# Autodesk Inventor assembly: 1400_DC Coil_V1
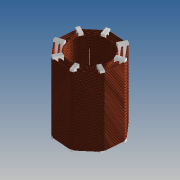
[picture p0: Inventor's stored thumbnail of the model, 180x180]
Saved by Autodesk Inventor 2020 (Build 240168000, 168)
## iProperties
Created: 2019-11-14
Part Number: 1400_DC Coil_V1
Document SubType Name: Assembly
Designer: RFLab
Author: RFLab
## Documents named in this file (6)
- C:\Users\RFLab\Dropbox\MPI Group Folder\MPS\Inventor_Parts\Parts Numbered - OSMPI\1xxx_Transmit Assembly\14xx_Bias Coils\1400_DC Coil_V1.iam
- C:\Users\RFLab\Dropbox\MPI Group Folder\MPS\Inventor_Parts\Parts Numbered - OSMPI\1xxx_Transmit Assembly\14xx_Bias Coils\1401A_Bias Coil Wire_V1.ipt
- C:\Users\RFLab\Dropbox\MPI Group Folder\MPS\Inventor_Parts\Parts Numbered - OSMPI\1xxx_Transmit Assembly\14xx_Bias Coils\1402_Bias Coil Spacer_V1.ipt
- C:\Users\RFLab\Dropbox\MPI Group Folder\MPS\Inventor_Parts\Parts Numbered - OSMPI\1xxx_Transmit Assembly\14xx_Bias Coils\1402B_Bias Coil Spacer_V1.ipt
- C:\Users\RFLab\Dropbox\MPI Group Folder\MPS\Inventor_Parts\Parts Numbered - OSMPI\1xxx_Transmit Assembly\14xx_Bias Coils\1401B_Bias Coil Wire_V1.ipt
- C:\Users\RFLab\Dropbox\MPI Group Folder\MPS\Inventor_Parts\Parts Numbered - OSMPI\1xxx_Transmit Assembly\14xx_Bias Coils\1401C_Bias Coil Wire_V1.ipt
## Components (5 placed, 5 different names)
1. 1401A_Bias Coil Wire_V1:1 — Mate:1, Angle:1, Mate:3, Mate:4, Mate:6, Mate:8
2. 1402_Bias Coil Spacer_V1:1 — Mate:4, Mate:5, Mate:7, Flush:1, Flush:2, Angle:3
3. 1401B_Bias Coil Wire_V1:1 — Mate:6, Mate:7, Angle:2, Angle:3, Angle:4
4. 1402B_Bias Coil Spacer_V1:1 — Mate:8, Flush:1, Angle:2, Flush:2, Mate:9, Mate:10
5. 1401C_Bias Coil Wire_V1:1 — Mate:9, Mate:10, Angle:4
## Relationships (15: Mate 9, Angle 4, Flush 2)
- Mate:1: 1401A_Bias Coil Wire_V1:1
- Angle:1 (0 deg): 1401A_Bias Coil Wire_V1:1
- Mate:3: 1401A_Bias Coil Wire_V1:1
- Mate:4: 1401A_Bias Coil Wire_V1:1 ↔ 1402_Bias Coil Spacer_V1:1
- Mate:5 (-3.45 mm): 1402_Bias Coil Spacer_V1:1
- Mate:6: 1401A_Bias Coil Wire_V1:1 ↔ 1401B_Bias Coil Wire_V1:1
- Mate:7 (0.45 mm): 1402_Bias Coil Spacer_V1:1 ↔ 1401B_Bias Coil Wire_V1:1
- Mate:8: 1401A_Bias Coil Wire_V1:1 ↔ 1402B_Bias Coil Spacer_V1:1
- Flush:1: 1402_Bias Coil Spacer_V1:1 ↔ 1402B_Bias Coil Spacer_V1:1
- Angle:2 (0 deg): 1401B_Bias Coil Wire_V1:1 ↔ 1402B_Bias Coil Spacer_V1:1
- Flush:2: 1402_Bias Coil Spacer_V1:1 ↔ 1402B_Bias Coil Spacer_V1:1
- Mate:9: 1402B_Bias Coil Spacer_V1:1 ↔ 1401C_Bias Coil Wire_V1:1
- Mate:10 (0.45 mm): 1402B_Bias Coil Spacer_V1:1 ↔ 1401C_Bias Coil Wire_V1:1
- Angle:3 (0 deg): 1402_Bias Coil Spacer_V1:1 ↔ 1401B_Bias Coil Wire_V1:1
- Angle:4 (0 deg): 1401B_Bias Coil Wire_V1:1 ↔ 1401C_Bias Coil Wire_V1:1
